# Autodesk Inventor assembly: Assembly1
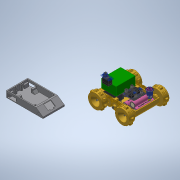
[picture p0: Inventor's stored thumbnail of the model, 180x180]
Saved by Autodesk Inventor 2020 (Build 240168000, 168)
## iProperties
Created: 2020-01-27
Part Number: Assembly1
Document SubType Name: Assembly
Designer: blep
Author: blep
## Documents named in this file (19)
- C:\Users\blep\Desktop\ScanBot\3d-model\Assembly1.iam
- C:\Users\blep\Desktop\ScanBot\3d-model\Tower Pro MG90S Micro servo\Tower Pro MG90S Micro servo.iam
- C:\Users\blep\Documents\Inventor\Content Center Files\R2020\pl-PL\AS 1427(08)\AS 1427 - M4 x 16(6) I.ipt
- C:\Users\blep\Desktop\ScanBot\3d-model\wheel.ipt
- C:\Users\blep\Desktop\ScanBot\3d-model\wheel_MIR.ipt
- C:\Users\blep\Desktop\ScanBot\3d-model\wheel_FRONT.ipt
- C:\Users\blep\Desktop\ScanBot\3d-model\wheel_FRONT_MIR.ipt
- C:\Users\blep\Desktop\ScanBot\3d-model\MG996R servo\MG_996R.iam
- C:\Users\blep\Desktop\ScanBot\3d-model\led on off push button\16mm-LED-Power-Button.iam
- C:\Users\blep\Desktop\ScanBot\3d-model\base.ipt
- C:\Users\blep\Documents\base-v2.ipt
- C:\Users\blep\Documents\small-gear-v2.ipt
- C:\Users\blep\Documents\small-gear-v2_MIR.ipt
- C:\Users\blep\Desktop\ScanBot\3d-model\EC11 encoder - long\EC11_Rotary_Encoder_Switched.ipt
- C:\Users\blep\Documents\small-gear-v2_CPY.ipt
- C:\Users\blep\Desktop\ScanBot\3d-model\18650 battery\18650.ipt
- C:\Users\blep\Documents\small-gear-v2_CPY_MIR.ipt
- C:\Users\blep\Desktop\ScanBot\3d-model\lm2596 buck converter\LM2596 DC-DC StepDown Converter v1.ipt
- C:\Users\blep\Documents\motherboard.ipt
## Components (27 placed, 18 different names)
1. MG_996R:1 [sub-assembly] — Równoległe:15, Równoległe:17, Zestawiające:12, Obrotowe:8
2. MG_996R:2 [sub-assembly] — Równoległe:15, Równoległe:16, Obrotowe:7, Zestawiające:11, Zestawiające:13
3. 16mm-LED-Power-Button:1 [sub-assembly]
4. base:1
5. base-v2:1 — Zestawiające:6, Zestawiające:9, Zestawiające:10, Obrotowe:1, Obrotowe:6, Obrotowe:2, Obrotowe:3, Równoległe:16, Równoległe:17, Zestawiające:11, Zestawiające:12, Zestawiające:13, Sztywne:1, Sztywne:2, Sztywne:3, Sztywne:4, Zestawiające:14, Styczny:3, Styczny:4, Styczny:5, Styczny:9, Sztywne:5, Sztywne:6
6. small-gear-v2:1 — Obrotowe:7
7. small-gear-v2_MIR:1 — Obrotowe:8
8. small-gear-v2_CPY:1 — Obrotowe:9
9. 18650:1 — Styczny:1, Równoległe:18, Zestawiające:14, Styczny:3
10. 18650:2 — Styczny:1, Równoległe:18, Styczny:4, Równoległe:20, Styczny:7, Styczny:8
11. 18650:3 — Styczny:2, Równoległe:19, Styczny:5, Równoległe:20, Styczny:7, Styczny:9
12. 18650:4 — Styczny:2, Równoległe:19, Styczny:8
13. EC11_Rotary_Encoder_Switched:1 — Sztywne:6, Obrotowe:10
14. EC11_Rotary_Encoder_Switched:2 — Sztywne:5, Obrotowe:9
15. small-gear-v2_CPY_MIR:1 — Obrotowe:10
16. LM2596 DC-DC StepDown Converter v1:1
17. LM2596 DC-DC StepDown Converter v1:2
18. motherboard:1
19. wheel:1 — Obrotowe:6
20. wheel_MIR:1 — Obrotowe:1
21. wheel_FRONT:1 — Obrotowe:3
22. wheel_FRONT_MIR:1 — Obrotowe:2
23. AS 1427 Z - Metryczny M4 x 16:8 — Sztywne:4
24. AS 1427 Z - Metryczny M4 x 16:9 — Sztywne:1
25. AS 1427 Z - Metryczny M4 x 16:10 — Sztywne:3
26. AS 1427 Z - Metryczny M4 x 16:13 — Sztywne:2
27. Tower Pro MG90S Micro servo:3 [sub-assembly]
## Relationships (35: RevoluteJoint 8, Tangent 8, Mate 7, Flush 6, WeldJoint 6)
- Zestawiające:6 [Mate]: base-v2:1
- Zestawiające:9 [Mate]: base-v2:1
- Zestawiające:10 [Mate]: base-v2:1
- Obrotowe:1 [RevoluteJoint] (-0.5 mm): base-v2:1 ↔ wheel_MIR:1
- Obrotowe:6 [RevoluteJoint] (0.5 mm): base-v2:1 ↔ wheel:1
- Obrotowe:2 [RevoluteJoint] (-0.5 mm): base-v2:1 ↔ wheel_FRONT_MIR:1
- Obrotowe:3 [RevoluteJoint] (0.5 mm): base-v2:1 ↔ wheel_FRONT:1
- Równoległe:15 [Flush]: MG_996R:1 ↔ MG_996R:2
- Równoległe:16 [Flush] (0.5 mm): MG_996R:2 ↔ base-v2:1
- Równoległe:17 [Flush] (0.5 mm): MG_996R:1 ↔ base-v2:1
- Obrotowe:7 [RevoluteJoint] (-0.2 mm): MG_996R:2 ↔ small-gear-v2:1
- Zestawiające:11 [Mate]: MG_996R:2 ↔ base-v2:1
- Zestawiające:12 [Mate]: MG_996R:1 ↔ base-v2:1
- Zestawiające:13 [Mate] (4.7 mm): MG_996R:2 ↔ base-v2:1
- Obrotowe:8 [RevoluteJoint] (-0.2 mm): MG_996R:1 ↔ small-gear-v2_MIR:1
- Sztywne:1 [WeldJoint]: base-v2:1 ↔ AS 1427 Z - Metryczny M4 x 16:9
- Sztywne:2 [WeldJoint]: base-v2:1 ↔ AS 1427 Z - Metryczny M4 x 16:13
- Sztywne:3 [WeldJoint]: base-v2:1 ↔ AS 1427 Z - Metryczny M4 x 16:10
- Sztywne:4 [WeldJoint]: base-v2:1 ↔ AS 1427 Z - Metryczny M4 x 16:8
- Styczny:1 [Tangent]: 18650:1 ↔ 18650:2
- Styczny:2 [Tangent]: 18650:3 ↔ 18650:4
- Równoległe:18 [Flush]: 18650:1 ↔ 18650:2
- Równoległe:19 [Flush]: 18650:3 ↔ 18650:4
- Zestawiające:14 [Mate] (7.5 mm): base-v2:1 ↔ 18650:1
- Styczny:3 [Tangent]: base-v2:1 ↔ 18650:1
- Styczny:4 [Tangent]: base-v2:1 ↔ 18650:2
- Styczny:5 [Tangent]: base-v2:1 ↔ 18650:3
- Równoległe:20 [Flush]: 18650:2 ↔ 18650:3
- Styczny:7 [Tangent]: 18650:2 ↔ 18650:3
- Styczny:8 [Tangent]: 18650:2 ↔ 18650:4
- Styczny:9 [Tangent] (0.5 mm): base-v2:1 ↔ 18650:3
- Sztywne:5 [WeldJoint]: base-v2:1 ↔ EC11_Rotary_Encoder_Switched:2
- Obrotowe:9 [RevoluteJoint] (16.7 mm): small-gear-v2_CPY:1 ↔ EC11_Rotary_Encoder_Switched:2
- Sztywne:6 [WeldJoint]: base-v2:1 ↔ EC11_Rotary_Encoder_Switched:1
- Obrotowe:10 [RevoluteJoint] (-16.7 mm): EC11_Rotary_Encoder_Switched:1 ↔ small-gear-v2_CPY_MIR:1
